# Autodesk Inventor assembly: Mx64_with_bearing_MIR1
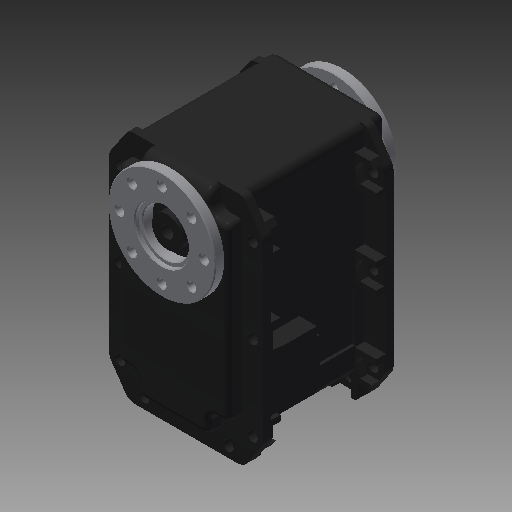
[picture p0: Inventor's stored thumbnail of the model, 512x512]
Saved by Autodesk Inventor 2018 (Build 220112000, 112)
## iProperties
Created: 2014-04-23
Part Number: Mx64_with_bearing_MIR1
Document SubType Name: Assembly
Designer: jaspe
Author: BitBots
## Documents named in this file (4)
- C:\Users\jaspe\bitbots_hardware\wolfgang\assembly\motors\MX64\Mx64_with_bearing_MIR1.iam
- C:\Users\jaspe\bitbots_hardware\wolfgang\assembly\motors\MX64\MX64_body_modified_MIR1.ipt
- C:\Users\jaspe\bitbots_hardware\wolfgang\assembly\motors\MX64\HN05-i1_MIR2.ipt
- C:\Users\jaspe\bitbots_hardware\wolfgang\assembly\motors\MX64\HN05-N101_MIR2.ipt
## Components (3 placed, 3 different names)
1. MX64_body_modified_MIR1:1 — Mate:1, Flush:2, Flush:1, Rotational:4, Rotational:5
2. HN05-i1_MIR2:1 — Rotational:4
3. HN05-N101_MIR2:1 — Rotational:5
## Relationships (5: Mate 2, RevoluteJoint 2, Flush 1)
- Mate:1: MX64_body_modified_MIR1:1
- Flush:2 [Mate]: MX64_body_modified_MIR1:1
- Flush:1: MX64_body_modified_MIR1:1
- Rotational:4 [RevoluteJoint]: MX64_body_modified_MIR1:1 ↔ HN05-i1_MIR2:1
- Rotational:5 [RevoluteJoint]: MX64_body_modified_MIR1:1 ↔ HN05-N101_MIR2:1
